# Autodesk Inventor assembly: Ensamblaje1
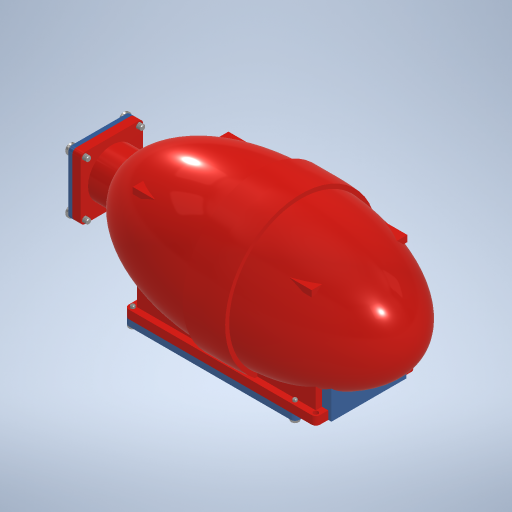
[picture p0: Inventor's stored thumbnail of the model, 512x512]
Saved by Autodesk Inventor 2023 (Build 270158000, 158)
## iProperties
Created: 2023-03-19
Part Number: Ensamblaje1
Document SubType Name: Assembly
Designer: sergi
Author: sergi
## Documents named in this file (7)
- C:\Users\sergi\OneDrive\Escritorio\Diseño submarino\Ensamblaje1.iam
- C:\Users\sergi\OneDrive\Escritorio\Diseño submarino\Submarino.ipt
- C:\Users\sergi\OneDrive\Escritorio\Diseño submarino\Capsula.ipt
- C:\Users\sergi\OneDrive\Escritorio\Diseño submarino\Tapa trasera.ipt
- C:\Users\sergi\OneDrive\Documentos\Inventor\Content Center Files\R2023\es-ES\GB_T 67\Screw GB_T 67 M2,5 x 8.ipt
- C:\Users\sergi\OneDrive\Escritorio\Diseño submarino\Tapa principal.ipt
- C:\Users\sergi\OneDrive\Documentos\Inventor\Content Center Files\R2023\es-ES\GB_T 67\Screw GB_T 67 M2 x 8.ipt
## Components (12 placed, 6 different names)
1. Submarino:1 — Rígido:1, De rotación:1, Rígido:2
2. Capsula:1 — Rígido:1
3. Tapa trasera:1 — De rotación:1, Coincidencia:23, Coincidencia:24, Coincidencia:25, Coincidencia:26, Coincidencia:27, Coincidencia:28, Coincidencia:29, Coincidencia:30
4. Screw GB/T 67 M2,5 x 8:3 — Coincidencia:23, Coincidencia:24
5. Screw GB/T 67 M2,5 x 8:2 — Coincidencia:27, Coincidencia:28
6. Screw GB/T 67 M2,5 x 8:1 — Coincidencia:29, Coincidencia:30
7. Tapa principal:1 — Rígido:2, Coincidencia:31, Coincidencia:32, Coincidencia:33, Coincidencia:34, Coincidencia:35, Coincidencia:36, Coincidencia:37, Coincidencia:38
8. Screw GB/T 67 M2 x 8:1 — Coincidencia:31, Coincidencia:32
9. Screw GB/T 67 M2 x 8:2 — Coincidencia:33, Coincidencia:34
10. Screw GB/T 67 M2 x 8:3 — Coincidencia:35, Coincidencia:36
11. Screw GB/T 67 M2 x 8:4 — Coincidencia:37, Coincidencia:38
12. Screw GB/T 67 M2,5 x 8:4 — Coincidencia:25, Coincidencia:26
## Relationships (19: Mate 16, WeldJoint 2, RevoluteJoint 1)
- Rígido:1 [WeldJoint]: Submarino:1 ↔ Capsula:1
- De rotación:1 [RevoluteJoint]: Submarino:1 ↔ Tapa trasera:1
- Rígido:2 [WeldJoint]: Submarino:1 ↔ Tapa principal:1
- Coincidencia:23 [Mate]: Tapa trasera:1 ↔ Screw GB/T 67 M2,5 x 8:3
- Coincidencia:24 [Mate]: Tapa trasera:1 ↔ Screw GB/T 67 M2,5 x 8:3
- Coincidencia:25 [Mate]: Tapa trasera:1 ↔ Screw GB/T 67 M2,5 x 8:4
- Coincidencia:26 [Mate]: Tapa trasera:1 ↔ Screw GB/T 67 M2,5 x 8:4
- Coincidencia:27 [Mate]: Tapa trasera:1 ↔ Screw GB/T 67 M2,5 x 8:2
- Coincidencia:28 [Mate]: Tapa trasera:1 ↔ Screw GB/T 67 M2,5 x 8:2
- Coincidencia:29 [Mate]: Tapa trasera:1 ↔ Screw GB/T 67 M2,5 x 8:1
- Coincidencia:30 [Mate]: Tapa trasera:1 ↔ Screw GB/T 67 M2,5 x 8:1
- Coincidencia:31 [Mate]: Tapa principal:1 ↔ Screw GB/T 67 M2 x 8:1
- Coincidencia:32 [Mate]: Tapa principal:1 ↔ Screw GB/T 67 M2 x 8:1
- Coincidencia:33 [Mate]: Tapa principal:1 ↔ Screw GB/T 67 M2 x 8:2
- Coincidencia:34 [Mate]: Tapa principal:1 ↔ Screw GB/T 67 M2 x 8:2
- Coincidencia:35 [Mate]: Tapa principal:1 ↔ Screw GB/T 67 M2 x 8:3
- Coincidencia:36 [Mate]: Tapa principal:1 ↔ Screw GB/T 67 M2 x 8:3
- Coincidencia:37 [Mate]: Tapa principal:1 ↔ Screw GB/T 67 M2 x 8:4
- Coincidencia:38 [Mate]: Tapa principal:1 ↔ Screw GB/T 67 M2 x 8:4
